# Autodesk Inventor assembly: Export chasis
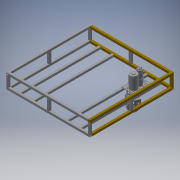
[picture p0: Inventor's stored thumbnail of the model, 180x180]
Saved by Autodesk Inventor 2019 (Build 230136000, 136)
## iProperties
Created: 2019-01-05
Part Number: Export chasis
Document SubType Name: Assembly
Designer: Jacob's Laptop
Author: Jacob's Laptop
## Documents named in this file (15)
- D:\Synthesis Robots\Epsilon\Export chasis.iam
- D:\Synthesis Robots\Epsilon\Chasis Long Length.ipt
- D:\Synthesis Robots\Epsilon\Chasis Short Length.ipt
- D:\Synthesis Robots\Epsilon\Chasis Hieght.ipt
- C:\Users\josh\Downloads\am-3009+Swerve+&+Steer+Rev+2016.iam
- C:\Users\josh\Downloads\Swerve & Steer Bot Rev 2.iam
- C:\Users\josh\Downloads\40-20 1-25 mod bevel gear pair.iam
- C:\Users\josh\Downloads\4 in HiGrip Wheel.iam
- C:\Users\josh\Downloads\20t 1-25mod bevel gear.ipt
- C:\Users\josh\Downloads\40t 1-25mod bevel gear.ipt
- C:\Users\josh\Downloads\375 Hex Output Shaft Rev 2.ipt
- C:\Users\josh\Downloads\375 E-klip - Mcm 97431A320_97431A320.ipt
- C:\Users\josh\Downloads\FR6ZZ-L Hex Bearing.ipt
- C:\Users\josh\Downloads\375 Hex Hub.ipt
- C:\Users\josh\Downloads\10-24 Hex Washer Rolling x 3-4_93882A213.ipt
## Components (38 placed, 21 different names)
1. Chasis Long Length:1 — Mate:1, Flush:1, Flush:2, Mate:2, Flush:3, Flush:4, Mate:3, Flush:5, Flush:6, Mate:6, Flush:12
2. 10-24 Hex Washer Rolling x 3-4_93882A213_15
3. 10-24 Hex Washer Rolling x 3-4_93882A213_16
4. 10-24 Hex Washer Rolling x 3-4_93882A213_17
5. 10-24 Hex Washer Rolling x 3-4_93882A213_18
6. 10-24 Hex Washer Rolling x 3-4_93882A213_19
7. 10-24 Hex Washer Rolling x 3-4_93882A213_20
8. Chasis Long Length:2 — Mate:4, Flush:7, Flush:8, Mate:5, Flush:9, Mate:7, Flush:13, Flush:14
9. Chasis Short Length:1 — Mate:2, Flush:3, Flush:4
10. Chasis Short Length:2 — Mate:3, Flush:5, Flush:6, Mate:4, Flush:7, Flush:8, Flush:10, Flush:11, Flush:24
11. Chasis Hieght:1 — Mate:1, Flush:1, Flush:2, Mate:11, Flush:21, Flush:22, Mate:13, Mate:17
12. Chasis Hieght:2 — Mate:6, Flush:11, Flush:12
13. Chasis Hieght:3 — Mate:5, Flush:9, Flush:10, Mate:15
14. Chasis Hieght:4 — Mate:7, Flush:13, Flush:14, Mate:19
15. FR6ZZ-L Hex Bearing_5 — Rotational:8, Mate:54
16. 375 E-klip - Mcm 97431A320_97431A320_22 — Rotational:6, Mate:55
17. FR6ZZ-L Hex Bearing_6 — Rotational:9, Mate:55
18. Chasis Long Length:3 — Mate:11, Flush:21, Flush:22, Mate:16, Flush:25
19. Chasis Long Length:4 — Mate:14, Mate:21, Flush:27, Mate:22, Flush:28, Mate:23, Flush:29, Mate:24, Flush:30
20. Chasis Short Length:3 — Mate:18, Flush:26, Mate:27
21. Chasis Short Length:4 — Mate:12, Flush:23, Mate:28
22. Chasis Hieght:5 — Mate:18, Flush:26, Mate:19
23. Chasis Hieght:6 — Mate:16, Flush:25, Mate:17
24. Chasis Hieght:7 — Mate:12, Flush:23, Mate:13
25. 375 Hex Hub_14 — Mate:50, Mate:51, Mate:52
26. Chasis Hieght:8 — Mate:14, Flush:24, Mate:15
27. Chasis Short Length:5 — Mate:21, Flush:27, Mate:25, Mate:27, Flush:32
28. Chasis Short Length:6 — Mate:22, Flush:28, Mate:25, Mate:31
29. Chasis Short Length:7 — Mate:23, Flush:29, Mate:26
30. Chasis Short Length:8 — Mate:24, Flush:30, Mate:26, Mate:28
31. 20t 1-25mod bevel gear_46 — Rotational:1
32. 40t 1-25mod bevel gear_47 — Mate:53, Mate:56, Mate:57, Mate:58, Mate:59
33. 375 Hex Output Shaft Rev 2_12 — Rotational:6, Mate:50, Mate:51, Mate:52, Mate:54, Mate:58, Mate:59
34. 375 E-klip - Mcm 97431A320_97431A320_23 — Mate:56, Mate:57
35. 40-20 1-25 mod bevel gear pair_8 [sub-assembly]
36. 4 in HiGrip Wheel_13 [sub-assembly] — Mate:53
37. Swerve & Steer Bot Rev 2_2 [sub-assembly] — Rotational:1, Rotational:8, Rotational:9
38. am-3009+Swerve+&+Steer+Rev+2016:1 [sub-assembly] — Mate:31, Flush:32
## Relationships (89: Mate 54, Flush 31, RevoluteJoint 4)
- Mate:1: Chasis Long Length:1 ↔ Chasis Hieght:1
- Flush:1: Chasis Long Length:1 ↔ Chasis Hieght:1
- Flush:2: Chasis Long Length:1 ↔ Chasis Hieght:1
- Mate:2: Chasis Long Length:1 ↔ Chasis Short Length:1
- Flush:3: Chasis Long Length:1 ↔ Chasis Short Length:1
- Flush:4: Chasis Long Length:1 ↔ Chasis Short Length:1
- Mate:3: Chasis Long Length:1 ↔ Chasis Short Length:2
- Flush:5: Chasis Long Length:1 ↔ Chasis Short Length:2
- Flush:6: Chasis Long Length:1 ↔ Chasis Short Length:2
- Mate:4: Chasis Long Length:2 ↔ Chasis Short Length:2
- Flush:7: Chasis Long Length:2 ↔ Chasis Short Length:2
- Flush:8: Chasis Long Length:2 ↔ Chasis Short Length:2
- Mate:5: Chasis Long Length:2 ↔ Chasis Hieght:3
- Flush:9: Chasis Long Length:2 ↔ Chasis Hieght:3
- Flush:10: Chasis Short Length:2 ↔ Chasis Hieght:3
- Mate:6: Chasis Long Length:1 ↔ Chasis Hieght:2
- Flush:11: Chasis Short Length:2 ↔ Chasis Hieght:2
- Flush:12: Chasis Long Length:1 ↔ Chasis Hieght:2
- Mate:7: Chasis Long Length:2 ↔ Chasis Hieght:4
- Flush:13: Chasis Long Length:2 ↔ Chasis Hieght:4
- Flush:14: Chasis Long Length:2 ↔ Chasis Hieght:4
- [Mate]: Chasis Long Length:3 ↔ Chasis Short Length:3
- [Flush]: Chasis Long Length:3 ↔ Chasis Short Length:3
- [Flush]: Chasis Long Length:3 ↔ Chasis Short Length:3
- [Mate]: Chasis Long Length:3 ↔ Chasis Short Length:4
- [Flush]: Chasis Long Length:3 ↔ Chasis Short Length:4
- [Flush]: Chasis Long Length:3 ↔ Chasis Short Length:4
- [Mate]: Chasis Long Length:4 ↔ Chasis Short Length:4
- [Flush]: Chasis Long Length:4 ↔ Chasis Short Length:4
- [Flush]: Chasis Long Length:4 ↔ Chasis Short Length:4
- Mate:11: Chasis Hieght:1 ↔ Chasis Long Length:3
- Flush:21: Chasis Hieght:1 ↔ Chasis Long Length:3
- Flush:22: Chasis Hieght:1 ↔ Chasis Long Length:3
- Mate:12: Chasis Short Length:4 ↔ Chasis Hieght:7
- Flush:23: Chasis Short Length:4 ↔ Chasis Hieght:7
- Mate:13 (349.25 mm): Chasis Hieght:1 ↔ Chasis Hieght:7
- Mate:14: Chasis Long Length:4 ↔ Chasis Hieght:8
- Flush:24: Chasis Short Length:2 ↔ Chasis Hieght:8
- Mate:15 (349.25 mm): Chasis Hieght:3 ↔ Chasis Hieght:8
- Mate:16: Chasis Long Length:3 ↔ Chasis Hieght:6
- Flush:25: Chasis Long Length:3 ↔ Chasis Hieght:6
- Mate:17 (349.25 mm): Chasis Hieght:1 ↔ Chasis Hieght:6
- Mate:18: Chasis Short Length:3 ↔ Chasis Hieght:5
- Flush:26: Chasis Short Length:3 ↔ Chasis Hieght:5
- Mate:19 (349.25 mm): Chasis Hieght:4 ↔ Chasis Hieght:5
- Mate:21: Chasis Long Length:4 ↔ Chasis Short Length:5
- Flush:27: Chasis Long Length:4 ↔ Chasis Short Length:5
- Mate:22: Chasis Long Length:4 ↔ Chasis Short Length:6
- Flush:28: Chasis Long Length:4 ↔ Chasis Short Length:6
- Mate:23: Chasis Long Length:4 ↔ Chasis Short Length:7
- Flush:29: Chasis Long Length:4 ↔ Chasis Short Length:7
- Mate:24: Chasis Long Length:4 ↔ Chasis Short Length:8
- Flush:30: Chasis Long Length:4 ↔ Chasis Short Length:8
- Mate:25 (101.6 mm): Chasis Short Length:5 ↔ Chasis Short Length:6
- Mate:26 (101.6 mm): Chasis Short Length:7 ↔ Chasis Short Length:8
- Mate:27 (76.2 mm): Chasis Short Length:3 ↔ Chasis Short Length:5
- Mate:28 (76.2 mm): Chasis Short Length:4 ↔ Chasis Short Length:8
- Mate:31: Chasis Short Length:6 ↔ am-3009+Swerve+&+Steer+Rev+2016:1
- Flush:32: Chasis Short Length:5 ↔ am-3009+Swerve+&+Steer+Rev+2016:1
- [Mate]: 10-24 Hex Washer Rolling x 3-4_93882A213_17 ↔ 4 in HiGrip Wheel_13
- [Mate]: 10-24 Hex Washer Rolling x 3-4_93882A213_16 ↔ 4 in HiGrip Wheel_13
- [Mate]: 375 Hex Hub_14 ↔ 4 in HiGrip Wheel_13
- Rotational:1 [RevoluteJoint]: 20t 1-25mod bevel gear_46 ↔ Swerve & Steer Bot Rev 2_2
- [Mate]: FR6ZZ-L Hex Bearing_6 ↔ 375 Hex Output Shaft Rev 2_12
- [Mate]: 10-24 Hex Washer Rolling x 3-4_93882A213_16 ↔ 375 Hex Hub_14
- [Mate]: 10-24 Hex Washer Rolling x 3-4_93882A213_16 ↔ 375 Hex Hub_14
- [Mate]: 10-24 Hex Washer Rolling x 3-4_93882A213_15 ↔ 375 Hex Hub_14
- [Mate]: 10-24 Hex Washer Rolling x 3-4_93882A213_15 ↔ 375 Hex Hub_14
- [Mate]: 10-24 Hex Washer Rolling x 3-4_93882A213_20 ↔ 375 Hex Hub_14
- [Mate]: 10-24 Hex Washer Rolling x 3-4_93882A213_20 ↔ 375 Hex Hub_14
- [Mate]: 10-24 Hex Washer Rolling x 3-4_93882A213_19 ↔ 375 Hex Hub_14
- [Mate]: 10-24 Hex Washer Rolling x 3-4_93882A213_19 ↔ 375 Hex Hub_14
- [Mate]: 10-24 Hex Washer Rolling x 3-4_93882A213_18 ↔ 375 Hex Hub_14
- [Mate]: 10-24 Hex Washer Rolling x 3-4_93882A213_18 ↔ 375 Hex Hub_14
- [Mate]: 10-24 Hex Washer Rolling x 3-4_93882A213_17 ↔ 375 Hex Hub_14
- [Mate]: 10-24 Hex Washer Rolling x 3-4_93882A213_17 ↔ 375 Hex Hub_14
- Rotational:6 [RevoluteJoint]: 375 E-klip - Mcm 97431A320_97431A320_22 ↔ 375 Hex Output Shaft Rev 2_12
- Rotational:8 [RevoluteJoint]: FR6ZZ-L Hex Bearing_5 ↔ Swerve & Steer Bot Rev 2_2
- Mate:50: 375 Hex Hub_14 ↔ 375 Hex Output Shaft Rev 2_12
- Mate:51: 375 Hex Hub_14 ↔ 375 Hex Output Shaft Rev 2_12
- Mate:52: 375 Hex Hub_14 ↔ 375 Hex Output Shaft Rev 2_12
- Mate:53: 40t 1-25mod bevel gear_47 ↔ 4 in HiGrip Wheel_13
- Mate:54: FR6ZZ-L Hex Bearing_5 ↔ 375 Hex Output Shaft Rev 2_12
- Rotational:9 [RevoluteJoint]: FR6ZZ-L Hex Bearing_6 ↔ Swerve & Steer Bot Rev 2_2
- Mate:55: 375 E-klip - Mcm 97431A320_97431A320_22 ↔ FR6ZZ-L Hex Bearing_6
- Mate:56: 40t 1-25mod bevel gear_47 ↔ 375 E-klip - Mcm 97431A320_97431A320_23
- Mate:57: 40t 1-25mod bevel gear_47 ↔ 375 E-klip - Mcm 97431A320_97431A320_23
- Mate:58: 40t 1-25mod bevel gear_47 ↔ 375 Hex Output Shaft Rev 2_12
- Mate:59: 40t 1-25mod bevel gear_47 ↔ 375 Hex Output Shaft Rev 2_12
## Named parameters: d21_d3 = 0 mm, d22_d4 = 0 mm, d23_d5 = 0 mm, d24_d6 = 0 mm, d25_d7 = 0 mm, d26_d8 = 0 mm, d27_d9 = 0 mm, d28_d10 = 0 mm, d29_d11 = 0 mm, d108_d9 = 0 mm, d109_d10 = 0 mm, d110_d11 = 0 mm, d111_d0 = 0 mm, d112_d1 = 0 mm, d113_d2 = 0 mm, d114_d3 = 0 mm, d115_d4 = 0 mm, d116_d5 = 0 mm, d117_d6 = 0 mm, d118_d7 = 0 mm, d119_d8 = 0 mm
